# Autodesk Inventor assembly: Samenstel waterkanon januari
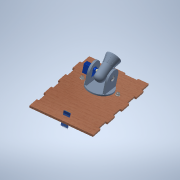
[picture p0: Inventor's stored thumbnail of the model, 180x180]
Saved by Autodesk Inventor 2021 (Build 250183000, 183)
## iProperties
Manager: Pierloot J.
Company: Emmaüs Bovenbouw Aalter
Created: 2017-06-09
Part Number: Samenstel waterkanon januari
Catalog Web Link: http://emmausbovenbouw.op-weg.be/
Vendor: Emmaüs Bovenbouw Aalter
Document SubType Name: Assembly
Designer: declercqs
Engineer: Declercq St.
Authority: Declercq St.
Title: Algemene Projecttitel
Author: declercqs
## Documents named in this file (13)
- F:\GIP 6EM\waterkannon\Samenstel waterkanon januari.iam
- F:\GIP 6EM\waterkannon\Waterkanon poging 3.ipt
- F:\GIP 6EM\waterkannon\Servomotor HTX900.ipt
- F:\GIP 6EM\waterkannon\Arm 1.ipt
- F:\GIP 6EM\waterkannon\Arm 3.ipt
- F:\GIP 6EM\waterkannon\Ball bearing 15mm.ipt
- F:\GIP 6EM\waterkannon\Tussenplaat bevestiging axiale lager.ipt
- F:\GIP 6EM\waterkannon\Onderste plaat bevestiging axiale lager.ipt
- F:\GIP 6EM\waterkannon\Axiale lager.ipt
- F:\GIP 6EM\waterkannon\Draaischijf waterkanon poging 2.0.ipt
- F:\GIP 6EM\Bevestigingen\Vijzen waterkanon.ipt
- F:\GIP 6EM\Bevestigingen\Moer Waterkanon.ipt
- F:\GIP 6EM\Assembly\Assembly HC-05.iam
## Components (15 placed, 12 different names)
1. Waterkanon poging 3:1 — Mate:29, Mate:31, Flush:57
2. Servomotor HTX900:1 — Mate:33, Mate:34, Mate:53, Flush:56
3. Servomotor HTX900:2 — Mate:38, Mate:39, Mate:45, Mate:47, Mate:69
4. Arm 1:1 — Mate:30, Mate:31, Mate:33, Mate:34, Flush:57
5. CSN 02 4740 81107:1 — Mate:38, Mate:56, Mate:57, Mate:58
6. Arm 3:1 — Mate:39
7. Ball bearing 15mm:1 — Mate:29, Mate:30, Mate:54, Mate:55
8. Tussenplaat bevestiging axiale lager:1 — Mate:46, Mate:48, Mate:52, Mate:58, Mate:68, Mate:70
9. Onderste plaat bevestiging axiale lager:1 — Mate:45, Mate:46, Mate:47, Mate:48, Mate:52, Mate:65, Mate:66, Mate:69, Mate:71, Mate:72
10. Draaischijf waterkanon poging 2.0:1 — Mate:53, Mate:54, Flush:56, Mate:55, Mate:56, Mate:57, Mate:67
11. Indented Hex Flange Head Machine Screw - Metric M5x0,8 x 25:1 — Mate:64, Mate:73
12. Indented Hex Flange Head Machine Screw - Metric M5x0,8 x 25:2 — Mate:63, Mate:74
13. BS 4183 - Metric M5:1 — Mate:63, Mate:66, Mate:71
14. BS 4183 - Metric M5:2 — Mate:64, Mate:65, Mate:72
15. Assembly HC-05:1 [sub-assembly] — Mate:67, Mate:68, Mate:70, Mate:73, Mate:74
## Relationships (32: Mate 30, Flush 2)
- Mate:29: Waterkanon poging 3:1 ↔ Ball bearing 15mm:1
- Mate:30: Arm 1:1 ↔ Ball bearing 15mm:1
- Mate:31: Waterkanon poging 3:1 ↔ Arm 1:1
- Mate:33: Servomotor HTX900:1 ↔ Arm 1:1
- Mate:34: Servomotor HTX900:1 ↔ Arm 1:1
- Mate:38 (5.5 mm): Servomotor HTX900:2 ↔ CSN 02 4740 81107:1
- Mate:39: Servomotor HTX900:2 ↔ Arm 3:1
- Mate:45: Servomotor HTX900:2 ↔ Onderste plaat bevestiging axiale lager:1
- Mate:46: Tussenplaat bevestiging axiale lager:1 ↔ Onderste plaat bevestiging axiale lager:1
- Mate:47: Servomotor HTX900:2 ↔ Onderste plaat bevestiging axiale lager:1
- Mate:48: Tussenplaat bevestiging axiale lager:1 ↔ Onderste plaat bevestiging axiale lager:1
- Mate:52: Tussenplaat bevestiging axiale lager:1 ↔ Onderste plaat bevestiging axiale lager:1
- Mate:53: Servomotor HTX900:1 ↔ Draaischijf waterkanon poging 2.0:1
- Mate:54: Ball bearing 15mm:1 ↔ Draaischijf waterkanon poging 2.0:1
- Flush:56: Servomotor HTX900:1 ↔ Draaischijf waterkanon poging 2.0:1
- Mate:55: Ball bearing 15mm:1 ↔ Draaischijf waterkanon poging 2.0:1
- Mate:56: CSN 02 4740 81107:1 ↔ Draaischijf waterkanon poging 2.0:1
- Mate:57 (0.3 mm): CSN 02 4740 81107:1 ↔ Draaischijf waterkanon poging 2.0:1
- Mate:58: CSN 02 4740 81107:1 ↔ Tussenplaat bevestiging axiale lager:1
- Flush:57: Waterkanon poging 3:1 ↔ Arm 1:1
- Mate:63: Indented Hex Flange Head Machine Screw - Metric M5x0,8 x 25:2 ↔ BS 4183 - Metric M5:1
- Mate:64: Indented Hex Flange Head Machine Screw - Metric M5x0,8 x 25:1 ↔ BS 4183 - Metric M5:2
- Mate:65: Onderste plaat bevestiging axiale lager:1 ↔ BS 4183 - Metric M5:2
- Mate:66: Onderste plaat bevestiging axiale lager:1 ↔ BS 4183 - Metric M5:1
- Mate:67: Draaischijf waterkanon poging 2.0:1 ↔ Assembly HC-05:1
- Mate:68: Tussenplaat bevestiging axiale lager:1 ↔ Assembly HC-05:1
- Mate:69: Servomotor HTX900:2 ↔ Onderste plaat bevestiging axiale lager:1
- Mate:70: Tussenplaat bevestiging axiale lager:1 ↔ Assembly HC-05:1
- Mate:71: Onderste plaat bevestiging axiale lager:1 ↔ BS 4183 - Metric M5:1
- Mate:72: Onderste plaat bevestiging axiale lager:1 ↔ BS 4183 - Metric M5:2
- Mate:73: Indented Hex Flange Head Machine Screw - Metric M5x0,8 x 25:1 ↔ Assembly HC-05:1
- Mate:74: Indented Hex Flange Head Machine Screw - Metric M5x0,8 x 25:2 ↔ Assembly HC-05:1
